# Autodesk Inventor assembly: 5mm to 8mm Coupler
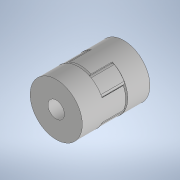
[picture p0: Inventor's stored thumbnail of the model, 180x180]
Saved by Autodesk Inventor 2022 (Build 260153000, 153)
## iProperties
Created: 2022-03-26
Part Number: 5mm to 8mm Coupler
Document SubType Name: Assembly
Designer: Nick
Author: Nick
## Documents named in this file (4)
- Y:\Projects\Bibble0\Hardware\5mm to 8mm Coupler.iam
- Y:\Projects\Bibble0\Hardware\Spider Coupler\Coupler - 5mm.ipt
- Y:\Projects\Bibble0\Hardware\Spider Coupler\Coupler - 8mm.ipt
- Y:\Projects\Bibble0\Hardware\Spider Coupler\Spider.ipt
## Components (3 placed, 3 different names)
1. Coupler - 5mm:1 — Insert:2, Tangent:2
2. Coupler - 8mm:1 — Insert:1, Tangent:1
3. Spider:1 — Insert:1, Insert:2, Tangent:1, Tangent:2
## Relationships (4: Insert 2, Tangent 2)
- Insert:1: Coupler - 8mm:1 ↔ Spider:1
- Insert:2: Coupler - 5mm:1 ↔ Spider:1
- Tangent:1: Coupler - 8mm:1 ↔ Spider:1
- Tangent:2: Coupler - 5mm:1 ↔ Spider:1
